# Autodesk Inventor assembly: Cerniera_definitiva
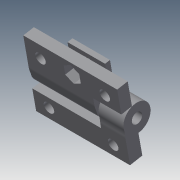
[picture p0: Inventor's stored thumbnail of the model, 180x180]
Saved by Autodesk Inventor 2019 (Build 230136000, 136)
## iProperties
Created: 2019-07-01
Part Number: Cerniera_definitiva
Document SubType Name: Assembly
Designer: giacomo
Author: giacomo
## Documents named in this file (3)
- D:\Hobby\Inventor\Prove 3D printer\Cerniera\Definitiva\Cerniera_definitiva.iam
- D:\Hobby\Inventor\Prove 3D printer\Cerniera\Definitiva\Cerniera_cov.ipt
- D:\Hobby\Inventor\Prove 3D printer\Cerniera\Definitiva\Cerniera_ins.ipt
## Components (2 placed, 2 different names)
1. Cerniera_cov:1 — Mate:1, Flush:1
2. Cerniera_ins:1 — Mate:1, Flush:1
## Relationships (2: Mate 1, Flush 1)
- Mate:1: Cerniera_cov:1 ↔ Cerniera_ins:1
- Flush:1: Cerniera_cov:1 ↔ Cerniera_ins:1
